# Autodesk Inventor assembly: 2021 Drive
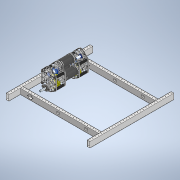
[picture p0: Inventor's stored thumbnail of the model, 180x180]
Saved by Autodesk Inventor 2021 (Build 250183000, 183)
## iProperties
Created: 2021-01-26
Part Number: 2021 Drive
Document SubType Name: Assembly
Designer: aidan
Author: aidan
## Documents named in this file (4)
- C:\Users\aidan\Desktop\T3 Robotics\CAD\2021 Specific Parts\2021 Drive.iam
- C:\Users\aidan\Desktop\T3 Robotics\CAD\Drive Train CAD\VerseFrame 30in.ipt
- C:\Users\aidan\Desktop\T3 Robotics\CAD\2021 Specific Parts\VerseFrame 2021 28in Drive.ipt
- C:\Users\aidan\Desktop\T3 Robotics\CAD\Drive Train CAD\WCP DS Gearbox.iam
## Components (6 placed, 3 different names)
1. VerseFrame 30in:1 — Flush:2, Flush:5, Mate:1
2. VerseFrame 30in:2 — Flush:3, Flush:5, Mate:2
3. VerseFrame 2021 28in Drive:1 — Flush:1, Flush:2, Flush:4, Mate:1, Mate:2, Mate:4
4. VerseFrame 2021 28in Drive:2 — Flush:1, Flush:3, Flush:4, Mate:3
5. WCP DS Gearbox:1 [sub-assembly] — Mate:4
6. WCP DS Gearbox:2 [sub-assembly] — Mate:3
## Relationships (9: Flush 5, Mate 4)
- Flush:1: VerseFrame 2021 28in Drive:1 ↔ VerseFrame 2021 28in Drive:2
- Flush:2: VerseFrame 30in:1 ↔ VerseFrame 2021 28in Drive:1
- Flush:3: VerseFrame 30in:2 ↔ VerseFrame 2021 28in Drive:2
- Flush:4: VerseFrame 2021 28in Drive:1 ↔ VerseFrame 2021 28in Drive:2
- Flush:5: VerseFrame 30in:1 ↔ VerseFrame 30in:2
- Mate:1: VerseFrame 30in:1 ↔ VerseFrame 2021 28in Drive:1
- Mate:2: VerseFrame 30in:2 ↔ VerseFrame 2021 28in Drive:1
- Mate:3: VerseFrame 2021 28in Drive:2 ↔ WCP DS Gearbox:2
- Mate:4: VerseFrame 2021 28in Drive:1 ↔ WCP DS Gearbox:1
